# Autodesk Inventor assembly: fc18-064
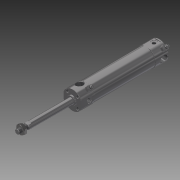
[picture p0: Inventor's stored thumbnail of the model, 180x180]
Saved by Autodesk Inventor 2018 (Build 220112000, 112)
## iProperties
Category: Pneumatics
Company: Autodesk Inc.
Created: 2017-11-24
Part Number: fc18-064
Catalog Web Link: http://firstchoicebyandymark.com/fc18-064
Document SubType Name: Assembly
Designer: Autodesk Inc.
Vendor: PHD Inc.
Author: Autodesk Inc.
Keywords: FIRSTChoice
## Documents named in this file (6)
- F:\FIRST 2018\FIRST 2018 FirstChoice\fc18-064_PneuCylinder.iam
- F:\FIRST 2018\FIRST 2018 FirstChoice\Parts\TUBE_OCG13_4x2_Open-Extend_.ipt
- F:\FIRST 2018\FIRST 2018 FirstChoice\Parts\HD_OCG13_4x2_Open-Extend.ipt
- F:\FIRST 2018\FIRST 2018 FirstChoice\Parts\PR_OCG1-3_4x2.ipt
- F:\FIRST 2018\FIRST 2018 FirstChoice\Parts\PN1972-015_NUT1_4-28-UNF.ipt
- F:\FIRST 2018\FIRST 2018 FirstChoice\Parts\CAP_OCG1-3_4.ipt
## Components (5 placed, 5 different names)
1. TUBE_OCG13_4x2_Open-Extend_:1 — Insert:1
2. HD_OCG13_4x2_Open-Extend:1 — Angle:1
3. PR_OCG1-3_4x2:1
4. PN1972-015_NUT1_4-28-UNF:1
5. CAP_OCG1-3_4:1 — Insert:1, Angle:1
## Relationships (2: Insert 1, Angle 1)
- Insert:1: TUBE_OCG13_4x2_Open-Extend_:1 ↔ CAP_OCG1-3_4:1
- Angle:1 (0 deg): HD_OCG13_4x2_Open-Extend:1 ↔ CAP_OCG1-3_4:1
